# Autodesk Inventor assembly: 000 Ensamblaje hw_DAA - PCB Sensor
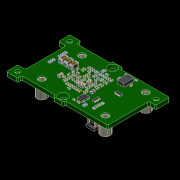
[picture p0: Inventor's stored thumbnail of the model, 180x180]
Saved by Autodesk Inventor 2018 (Build 220112000, 112)
## iProperties
Created: 2024-03-13
Part Number: 000 Ensamblaje hw_DAA - PCB Sensor
Document SubType Name: Assembly
Designer: cda1
Author: cda1
## Documents named in this file (15)
- C:\Users\cda1\Git\DAA\items\hw_DAA\variants\BASIC\3d\000 Ensamblaje hw_DAA - PCB Sensor.iam
- C:\Users\cda1\Git\DAA\items\hw_DAA\3d\hw_DAA - PCB Sensor.ipt
- C:\Users\cda1\Git\DAA\items\_accessories\Componentes PCB\Resistencias\3d_Panasonic\3d\ERJ-2RKF1002X.ipt
- C:\Users\cda1\Git\DAA\items\_accessories\Componentes PCB\Capacitadores\3d_TDK\3d\CGA2B3X7R1H104K050BD.ipt
- C:\Users\cda1\Git\DAA\items\_accessories\Componentes PCB\Condensadores\3d-Murata\3d\GRT188R61C106KE13D\GRT188R61C106KE13D.ipt
- C:\Users\cda1\Git\DAA\items\_accessories\Sensores imagen\3d_Sony\3d\IMX296LQR-C\IMX296LQR-C.ipt
- C:\Users\cda1\Git\DAA\items\_accessories\Componentes PCB\IMU\3d_Bosch\3d\BMI088.ipt
- C:\Users\cda1\Git\DAA\items\_accessories\Componentes PCB\Capacitadores\3d_Murata Electronics\3d\GRT31CC81C226KE01L.ipt
- C:\Users\cda1\Git\DAA\items\_accessories\Componentes PCB\Clock\3d_SiTime\3d\SiT8008BI-22-18E-37.125000G\SiT8008BI-22-18E-37.125000G.ipt
- C:\Users\cda1\Git\DAA\items\_accessories\Componentes PCB\Capacitadores\3d_Murata Electronics\3d\GRT188C81A106ME13D.ipt
- C:\Users\cda1\Git\DAA\items\_accessories\Componentes PCB\Resistencias\3d_Genérico\RESC-0402.ipt
- C:\Users\cda1\Git\DAA\items\_accessories\Componentes PCB\Resistencias\3d_Panasonic\3d\ERJ-2GE0R00X.ipt
- C:\Users\cda1\Git\DAA\items\_accessories\Componentes PCB\Elementos mecanicos soldables\3d_Wurth Electronics\3d\WA-SMST\9774050943\9774050943.ipt
- C:\Users\cda1\Git\DAA\items\_accessories\Componentes PCB\Conectores\3d_Amphenol Communications\SFW15S-2STE1LF\SFW15S-2STE1LF.ipt
- C:\Users\cda1\Git\DAA\items\_accessories\Componentes PCB\Diodos\3d_ST Microelectronics\HSP051-4M10\HSP051-4M10.ipt
## Components (113 placed, 14 different names)
1. hw_DAA - PCB Sensor:1 — Coincidencia:6, Coincidencia:7, Coincidencia:8, Coincidencia:9, Coincidencia:10, Coincidencia:11, Coincidencia:12, Coincidencia:13, Coincidencia:14, Coincidencia:15, Coincidencia:16, Coincidencia:17, Coincidencia:18, Coincidencia:19, Coincidencia:20, Coincidencia:21, Coincidencia:22, Coincidencia:23, Coincidencia:24, Coincidencia:25, Coincidencia:26, Coincidencia:27, Coincidencia:28, Coincidencia:29, Coincidencia:30, Coincidencia:32, Coincidencia:33, Coincidencia:34, Coincidencia:35, Coincidencia:36, Coincidencia:37, Coincidencia:38, Coincidencia:39, Coincidencia:40, Coincidencia:41, Coincidencia:42, Coincidencia:43, Coincidencia:44, Coincidencia:45, Coincidencia:46, Coincidencia:47, Coincidencia:48, Coincidencia:49, Coincidencia:50, Coincidencia:51, Coincidencia:52, Coincidencia:53, Coincidencia:54, Coincidencia:55, Coincidencia:56, Coincidencia:57, Coincidencia:58, Coincidencia:59, Coincidencia:60, Coincidencia:61, Coincidencia:62, Coincidencia:63, Coincidencia:64, Coincidencia:65, Coincidencia:66, Coincidencia:67, Coincidencia:68, Coincidencia:71, Coincidencia:72, Coincidencia:73, Coincidencia:74, Coincidencia:75, Coincidencia:76, Coincidencia:77, Coincidencia:78, Coincidencia:79, Coincidencia:80, Coincidencia:81, Coincidencia:82, Coincidencia:84, Coincidencia:85, Coincidencia:86, Coincidencia:87, Coincidencia:88, Coincidencia:90, Coincidencia:91, Coincidencia:92, Coincidencia:93, Coincidencia:94, Coincidencia:95, Coincidencia:96, Coincidencia:97, Coincidencia:98, Coincidencia:99, Coincidencia:100, Coincidencia:101, Coincidencia:102, Coincidencia:103, Coincidencia:104, Coincidencia:105, Coincidencia:106, Coincidencia:107, Coincidencia:108, Coincidencia:111, Coincidencia:112, Coincidencia:113, Coincidencia:114, Coincidencia:116, Coincidencia:117, Coincidencia:118, Coincidencia:121, Coincidencia:122, Coincidencia:123, Coincidencia:124, Coincidencia:125, Coincidencia:126, Coincidencia:127, Coincidencia:128, Ángulo:3, Ángulo:5, Ángulo:6, Ángulo:7, Ángulo:8, Coincidencia:129, Ángulo:9, Coincidencia:130, Coincidencia:131, Ángulo:10
2. ERJ-2RKF1002X:1 — Coincidencia:6
3. ERJ-2RKF1002X:2 — Coincidencia:7
4. ERJ-2RKF1002X:3 — Coincidencia:18
5. ERJ-2RKF1002X:4 — Coincidencia:17
6. ERJ-2RKF1002X:5 — Coincidencia:16
7. ERJ-2RKF1002X:6 — Coincidencia:15
8. ERJ-2RKF1002X:7 — Coincidencia:14
9. ERJ-2RKF1002X:8 — Coincidencia:13
10. ERJ-2RKF1002X:9 — Coincidencia:12
11. ERJ-2RKF1002X:10 — Coincidencia:11
12. ERJ-2RKF1002X:11 — Coincidencia:10
13. ERJ-2RKF1002X:12 — Coincidencia:9
14. ERJ-2RKF1002X:13 — Coincidencia:8
15. ERJ-2RKF1002X:14 — Coincidencia:19
16. CGA2B3X7R1H104K050BD:1 — Coincidencia:20, Ángulo:6
17. CGA2B3X7R1H104K050BD:2 — Coincidencia:21, Ángulo:7
18. CGA2B3X7R1H104K050BD:3 — Coincidencia:22
19. CGA2B3X7R1H104K050BD:4 — Coincidencia:23, Ángulo:5
20. CGA2B3X7R1H104K050BD:5 — Coincidencia:24
21. CGA2B3X7R1H104K050BD:6 — Coincidencia:25
22. CGA2B3X7R1H104K050BD:7 — Coincidencia:26
23. CGA2B3X7R1H104K050BD:8 — Coincidencia:28
24. CGA2B3X7R1H104K050BD:9 — Coincidencia:29
25. CGA2B3X7R1H104K050BD:10 — Coincidencia:30, Ángulo:8
26. CGA2B3X7R1H104K050BD:11 — Coincidencia:27
27. CGA2B3X7R1H104K050BD:13 — Coincidencia:32
28. CGA2B3X7R1H104K050BD:14 — Coincidencia:33
29. CGA2B3X7R1H104K050BD:15 — Coincidencia:34
30. CGA2B3X7R1H104K050BD:16 — Coincidencia:35
31. CGA2B3X7R1H104K050BD:17 — Coincidencia:36
32. CGA2B3X7R1H104K050BD:18 — Coincidencia:37
33. CGA2B3X7R1H104K050BD:19 — Coincidencia:38
34. CGA2B3X7R1H104K050BD:20 — Coincidencia:39
35. CGA2B3X7R1H104K050BD:21 — Coincidencia:40
36. CGA2B3X7R1H104K050BD:22 — Coincidencia:41
37. CGA2B3X7R1H104K050BD:23 — Coincidencia:42
38. CGA2B3X7R1H104K050BD:24 — Coincidencia:43
39. CGA2B3X7R1H104K050BD:25 — Coincidencia:44
40. CGA2B3X7R1H104K050BD:26 — Coincidencia:45
41. CGA2B3X7R1H104K050BD:27 — Coincidencia:46
42. CGA2B3X7R1H104K050BD:28 — Coincidencia:47
43. CGA2B3X7R1H104K050BD:29 — Coincidencia:48
44. CGA2B3X7R1H104K050BD:30 — Coincidencia:51
45. CGA2B3X7R1H104K050BD:31 — Coincidencia:52
46. CGA2B3X7R1H104K050BD:32 — Coincidencia:53
47. CGA2B3X7R1H104K050BD:33 — Coincidencia:68
48. CGA2B3X7R1H104K050BD:34 — Coincidencia:67
49. CGA2B3X7R1H104K050BD:35 — Coincidencia:66
50. CGA2B3X7R1H104K050BD:38 — Coincidencia:62
51. CGA2B3X7R1H104K050BD:39 — Coincidencia:63
52. CGA2B3X7R1H104K050BD:40 — Coincidencia:64
53. CGA2B3X7R1H104K050BD:41 — Coincidencia:65
54. CGA2B3X7R1H104K050BD:42 — Coincidencia:61
55. CGA2B3X7R1H104K050BD:43 — Coincidencia:60
56. CGA2B3X7R1H104K050BD:44 — Coincidencia:59
57. CGA2B3X7R1H104K050BD:45 — Coincidencia:58
58. CGA2B3X7R1H104K050BD:46 — Coincidencia:54
59. CGA2B3X7R1H104K050BD:47 — Coincidencia:55
60. CGA2B3X7R1H104K050BD:48 — Coincidencia:49
61. CGA2B3X7R1H104K050BD:49 — Coincidencia:50
62. CGA2B3X7R1H104K050BD:50 — Coincidencia:56
63. CGA2B3X7R1H104K050BD:51 — Coincidencia:57
64. CGA2B3X7R1H104K050BD:52 — Coincidencia:71
65. CGA2B3X7R1H104K050BD:53 — Coincidencia:72
66. CGA2B3X7R1H104K050BD:54 — Coincidencia:73
67. CGA2B3X7R1H104K050BD:55 — Coincidencia:74
68. CGA2B3X7R1H104K050BD:56 — Coincidencia:75
69. CGA2B3X7R1H104K050BD:57 — Coincidencia:76
70. CGA2B3X7R1H104K050BD:58 — Coincidencia:77
71. CGA2B3X7R1H104K050BD:59 — Coincidencia:78
72. GRT188R61C106KE13D:1 — Coincidencia:79
73. GRT188R61C106KE13D:2 — Coincidencia:80
74. GRT188R61C106KE13D:3 — Coincidencia:81
75. GRT188R61C106KE13D:4 — Coincidencia:82
76. IMX296LQR-C:1 — Coincidencia:84
77. BMI088:1 — Coincidencia:85
78. GRT31CC81C226KE01L:1 — Coincidencia:86
79. GRT31CC81C226KE01L:2 — Coincidencia:87
80. SiT8008BI-22-18E-37.125000G:1 — Coincidencia:88
81. ERJ-2RKF1002X:16 — Coincidencia:90, Ángulo:1
82. ERJ-2RKF1002X:17 — Coincidencia:91, Ángulo:1, Ángulo:2
83. ERJ-2RKF1002X:18 — Coincidencia:92, Ángulo:2
84. ERJ-2RKF1002X:19 — Coincidencia:94
85. ERJ-2RKF1002X:20 — Coincidencia:93
86. CGA2B3X7R1H104K050BD:60 — Coincidencia:95
87. CGA2B3X7R1H104K050BD:61 — Coincidencia:96
88. CGA2B3X7R1H104K050BD:62 — Coincidencia:97
89. GRT188C81A106ME13D:1 — Coincidencia:98
90. GRT31CC81C226KE01L:3 — Coincidencia:99, Ángulo:3
91. ERJ-2RKF1002X:21 — Coincidencia:100
92. ERJ-2RKF1002X:22 — Coincidencia:101
93. CGA2B3X7R1H104K050BD:63 — Coincidencia:102
94. CGA2B3X7R1H104K050BD:64 — Coincidencia:103
95. RESC-0402:1 — Coincidencia:104
96. ERJ-2GE0R00X:1 — Coincidencia:105
97. RESC-0402:2 — Coincidencia:106
98. CGA2B3X7R1H104K050BD:65 — Coincidencia:108
99. CGA2B3X7R1H104K050BD:66 — Coincidencia:107
100. ERJ-2RKF1002X:25 — Coincidencia:118
101. ERJ-2RKF1002X:26 — Coincidencia:117
102. ERJ-2RKF1002X:27 — Coincidencia:116
103. ERJ-2RKF1002X:29 — Coincidencia:114
104. ERJ-2RKF1002X:30 — Coincidencia:113
105. ERJ-2RKF1002X:31 — Coincidencia:112
106. ERJ-2RKF1002X:32 — Coincidencia:111
107. 9774050943:1 — Coincidencia:123, Coincidencia:124
108. 9774050943:2 — Coincidencia:121, Coincidencia:125
109. 9774050943:3 — Coincidencia:122, Coincidencia:126
110. 9774050943:4 — Coincidencia:127, Coincidencia:128
111. SFW15S-2STE1LF:1 — Coincidencia:129, Ángulo:9
112. HSP051-4M10:1 — Coincidencia:130
113. HSP051-4M10:2 — Coincidencia:131, Ángulo:10
## Relationships (125: Mate 116, Angle 9)
- Coincidencia:6 [Mate]: hw_DAA - PCB Sensor:1 ↔ ERJ-2RKF1002X:1
- Coincidencia:7 [Mate]: hw_DAA - PCB Sensor:1 ↔ ERJ-2RKF1002X:2
- Coincidencia:8 [Mate]: hw_DAA - PCB Sensor:1 ↔ ERJ-2RKF1002X:13
- Coincidencia:9 [Mate]: hw_DAA - PCB Sensor:1 ↔ ERJ-2RKF1002X:12
- Coincidencia:10 [Mate]: hw_DAA - PCB Sensor:1 ↔ ERJ-2RKF1002X:11
- Coincidencia:11 [Mate]: hw_DAA - PCB Sensor:1 ↔ ERJ-2RKF1002X:10
- Coincidencia:12 [Mate]: hw_DAA - PCB Sensor:1 ↔ ERJ-2RKF1002X:9
- Coincidencia:13 [Mate]: hw_DAA - PCB Sensor:1 ↔ ERJ-2RKF1002X:8
- Coincidencia:14 [Mate]: hw_DAA - PCB Sensor:1 ↔ ERJ-2RKF1002X:7
- Coincidencia:15 [Mate]: hw_DAA - PCB Sensor:1 ↔ ERJ-2RKF1002X:6
- Coincidencia:16 [Mate]: hw_DAA - PCB Sensor:1 ↔ ERJ-2RKF1002X:5
- Coincidencia:17 [Mate]: hw_DAA - PCB Sensor:1 ↔ ERJ-2RKF1002X:4
- Coincidencia:18 [Mate]: hw_DAA - PCB Sensor:1 ↔ ERJ-2RKF1002X:3
- Coincidencia:19 [Mate]: hw_DAA - PCB Sensor:1 ↔ ERJ-2RKF1002X:14
- Coincidencia:20 [Mate]: hw_DAA - PCB Sensor:1 ↔ CGA2B3X7R1H104K050BD:1
- Coincidencia:21 [Mate]: hw_DAA - PCB Sensor:1 ↔ CGA2B3X7R1H104K050BD:2
- Coincidencia:22 [Mate]: hw_DAA - PCB Sensor:1 ↔ CGA2B3X7R1H104K050BD:3
- Coincidencia:23 [Mate]: hw_DAA - PCB Sensor:1 ↔ CGA2B3X7R1H104K050BD:4
- Coincidencia:24 [Mate]: hw_DAA - PCB Sensor:1 ↔ CGA2B3X7R1H104K050BD:5
- Coincidencia:25 [Mate]: hw_DAA - PCB Sensor:1 ↔ CGA2B3X7R1H104K050BD:6
- Coincidencia:26 [Mate]: hw_DAA - PCB Sensor:1 ↔ CGA2B3X7R1H104K050BD:7
- Coincidencia:27 [Mate]: hw_DAA - PCB Sensor:1 ↔ CGA2B3X7R1H104K050BD:11
- Coincidencia:28 [Mate]: hw_DAA - PCB Sensor:1 ↔ CGA2B3X7R1H104K050BD:8
- Coincidencia:29 [Mate]: hw_DAA - PCB Sensor:1 ↔ CGA2B3X7R1H104K050BD:9
- Coincidencia:30 [Mate]: hw_DAA - PCB Sensor:1 ↔ CGA2B3X7R1H104K050BD:10
- Coincidencia:32 [Mate]: hw_DAA - PCB Sensor:1 ↔ CGA2B3X7R1H104K050BD:13
- Coincidencia:33 [Mate]: hw_DAA - PCB Sensor:1 ↔ CGA2B3X7R1H104K050BD:14
- Coincidencia:34 [Mate]: hw_DAA - PCB Sensor:1 ↔ CGA2B3X7R1H104K050BD:15
- Coincidencia:35 [Mate]: hw_DAA - PCB Sensor:1 ↔ CGA2B3X7R1H104K050BD:16
- Coincidencia:36 [Mate]: hw_DAA - PCB Sensor:1 ↔ CGA2B3X7R1H104K050BD:17
- Coincidencia:37 [Mate]: hw_DAA - PCB Sensor:1 ↔ CGA2B3X7R1H104K050BD:18
- Coincidencia:38 [Mate]: hw_DAA - PCB Sensor:1 ↔ CGA2B3X7R1H104K050BD:19
- Coincidencia:39 [Mate]: hw_DAA - PCB Sensor:1 ↔ CGA2B3X7R1H104K050BD:20
- Coincidencia:40 [Mate]: hw_DAA - PCB Sensor:1 ↔ CGA2B3X7R1H104K050BD:21
- Coincidencia:41 [Mate]: hw_DAA - PCB Sensor:1 ↔ CGA2B3X7R1H104K050BD:22
- Coincidencia:42 [Mate]: hw_DAA - PCB Sensor:1 ↔ CGA2B3X7R1H104K050BD:23
- Coincidencia:43 [Mate]: hw_DAA - PCB Sensor:1 ↔ CGA2B3X7R1H104K050BD:24
- Coincidencia:44 [Mate]: hw_DAA - PCB Sensor:1 ↔ CGA2B3X7R1H104K050BD:25
- Coincidencia:45 [Mate]: hw_DAA - PCB Sensor:1 ↔ CGA2B3X7R1H104K050BD:26
- Coincidencia:46 [Mate]: hw_DAA - PCB Sensor:1 ↔ CGA2B3X7R1H104K050BD:27
- Coincidencia:47 [Mate]: hw_DAA - PCB Sensor:1 ↔ CGA2B3X7R1H104K050BD:28
- Coincidencia:48 [Mate]: hw_DAA - PCB Sensor:1 ↔ CGA2B3X7R1H104K050BD:29
- Coincidencia:49 [Mate]: hw_DAA - PCB Sensor:1 ↔ CGA2B3X7R1H104K050BD:48
- Coincidencia:50 [Mate]: hw_DAA - PCB Sensor:1 ↔ CGA2B3X7R1H104K050BD:49
- Coincidencia:51 [Mate]: hw_DAA - PCB Sensor:1 ↔ CGA2B3X7R1H104K050BD:30
- Coincidencia:52 [Mate]: hw_DAA - PCB Sensor:1 ↔ CGA2B3X7R1H104K050BD:31
- Coincidencia:53 [Mate]: hw_DAA - PCB Sensor:1 ↔ CGA2B3X7R1H104K050BD:32
- Coincidencia:54 [Mate]: hw_DAA - PCB Sensor:1 ↔ CGA2B3X7R1H104K050BD:46
- Coincidencia:55 [Mate]: hw_DAA - PCB Sensor:1 ↔ CGA2B3X7R1H104K050BD:47
- Coincidencia:56 [Mate]: hw_DAA - PCB Sensor:1 ↔ CGA2B3X7R1H104K050BD:50
- Coincidencia:57 [Mate]: hw_DAA - PCB Sensor:1 ↔ CGA2B3X7R1H104K050BD:51
- Coincidencia:58 [Mate]: hw_DAA - PCB Sensor:1 ↔ CGA2B3X7R1H104K050BD:45
- Coincidencia:59 [Mate]: hw_DAA - PCB Sensor:1 ↔ CGA2B3X7R1H104K050BD:44
- Coincidencia:60 [Mate]: hw_DAA - PCB Sensor:1 ↔ CGA2B3X7R1H104K050BD:43
- Coincidencia:61 [Mate]: hw_DAA - PCB Sensor:1 ↔ CGA2B3X7R1H104K050BD:42
- Coincidencia:62 [Mate]: hw_DAA - PCB Sensor:1 ↔ CGA2B3X7R1H104K050BD:38
- Coincidencia:63 [Mate]: hw_DAA - PCB Sensor:1 ↔ CGA2B3X7R1H104K050BD:39
- Coincidencia:64 [Mate]: hw_DAA - PCB Sensor:1 ↔ CGA2B3X7R1H104K050BD:40
- Coincidencia:65 [Mate]: hw_DAA - PCB Sensor:1 ↔ CGA2B3X7R1H104K050BD:41
- Coincidencia:66 [Mate]: hw_DAA - PCB Sensor:1 ↔ CGA2B3X7R1H104K050BD:35
- Coincidencia:67 [Mate]: hw_DAA - PCB Sensor:1 ↔ CGA2B3X7R1H104K050BD:34
- Coincidencia:68 [Mate]: hw_DAA - PCB Sensor:1 ↔ CGA2B3X7R1H104K050BD:33
- Coincidencia:71 [Mate]: hw_DAA - PCB Sensor:1 ↔ CGA2B3X7R1H104K050BD:52
- Coincidencia:72 [Mate]: hw_DAA - PCB Sensor:1 ↔ CGA2B3X7R1H104K050BD:53
- Coincidencia:73 [Mate]: hw_DAA - PCB Sensor:1 ↔ CGA2B3X7R1H104K050BD:54
- Coincidencia:74 [Mate]: hw_DAA - PCB Sensor:1 ↔ CGA2B3X7R1H104K050BD:55
- Coincidencia:75 [Mate]: hw_DAA - PCB Sensor:1 ↔ CGA2B3X7R1H104K050BD:56
- Coincidencia:76 [Mate]: hw_DAA - PCB Sensor:1 ↔ CGA2B3X7R1H104K050BD:57
- Coincidencia:77 [Mate]: hw_DAA - PCB Sensor:1 ↔ CGA2B3X7R1H104K050BD:58
- Coincidencia:78 [Mate]: hw_DAA - PCB Sensor:1 ↔ CGA2B3X7R1H104K050BD:59
- Coincidencia:79 [Mate]: hw_DAA - PCB Sensor:1 ↔ GRT188R61C106KE13D:1
- Coincidencia:80 [Mate]: hw_DAA - PCB Sensor:1 ↔ GRT188R61C106KE13D:2
- Coincidencia:81 [Mate]: hw_DAA - PCB Sensor:1 ↔ GRT188R61C106KE13D:3
- Coincidencia:82 [Mate]: hw_DAA - PCB Sensor:1 ↔ GRT188R61C106KE13D:4
- Coincidencia:84 [Mate]: hw_DAA - PCB Sensor:1 ↔ IMX296LQR-C:1
- Coincidencia:85 [Mate]: hw_DAA - PCB Sensor:1 ↔ BMI088:1
- Coincidencia:86 [Mate]: hw_DAA - PCB Sensor:1 ↔ GRT31CC81C226KE01L:1
- Coincidencia:87 [Mate]: hw_DAA - PCB Sensor:1 ↔ GRT31CC81C226KE01L:2
- Coincidencia:88 [Mate]: hw_DAA - PCB Sensor:1 ↔ SiT8008BI-22-18E-37.125000G:1
- Coincidencia:90 [Mate]: hw_DAA - PCB Sensor:1 ↔ ERJ-2RKF1002X:16
- Coincidencia:91 [Mate]: hw_DAA - PCB Sensor:1 ↔ ERJ-2RKF1002X:17
- Coincidencia:92 [Mate]: hw_DAA - PCB Sensor:1 ↔ ERJ-2RKF1002X:18
- Coincidencia:93 [Mate]: hw_DAA - PCB Sensor:1 ↔ ERJ-2RKF1002X:20
- Coincidencia:94 [Mate]: hw_DAA - PCB Sensor:1 ↔ ERJ-2RKF1002X:19
- Coincidencia:95 [Mate]: hw_DAA - PCB Sensor:1 ↔ CGA2B3X7R1H104K050BD:60
- Coincidencia:96 [Mate]: hw_DAA - PCB Sensor:1 ↔ CGA2B3X7R1H104K050BD:61
- Coincidencia:97 [Mate]: hw_DAA - PCB Sensor:1 ↔ CGA2B3X7R1H104K050BD:62
- Coincidencia:98 [Mate]: hw_DAA - PCB Sensor:1 ↔ GRT188C81A106ME13D:1
- Coincidencia:99 [Mate]: hw_DAA - PCB Sensor:1 ↔ GRT31CC81C226KE01L:3
- Coincidencia:100 [Mate]: hw_DAA - PCB Sensor:1 ↔ ERJ-2RKF1002X:21
- Coincidencia:101 [Mate]: hw_DAA - PCB Sensor:1 ↔ ERJ-2RKF1002X:22
- Coincidencia:102 [Mate]: hw_DAA - PCB Sensor:1 ↔ CGA2B3X7R1H104K050BD:63
- Coincidencia:103 [Mate]: hw_DAA - PCB Sensor:1 ↔ CGA2B3X7R1H104K050BD:64
- Coincidencia:104 [Mate]: hw_DAA - PCB Sensor:1 ↔ RESC-0402:1
- Coincidencia:105 [Mate]: hw_DAA - PCB Sensor:1 ↔ ERJ-2GE0R00X:1
- Coincidencia:106 [Mate]: hw_DAA - PCB Sensor:1 ↔ RESC-0402:2
- Coincidencia:107 [Mate]: hw_DAA - PCB Sensor:1 ↔ CGA2B3X7R1H104K050BD:66
- Coincidencia:108 [Mate]: hw_DAA - PCB Sensor:1 ↔ CGA2B3X7R1H104K050BD:65
- Coincidencia:111 [Mate]: hw_DAA - PCB Sensor:1 ↔ ERJ-2RKF1002X:32
- Coincidencia:112 [Mate]: hw_DAA - PCB Sensor:1 ↔ ERJ-2RKF1002X:31
- Coincidencia:113 [Mate]: hw_DAA - PCB Sensor:1 ↔ ERJ-2RKF1002X:30
- Coincidencia:114 [Mate]: hw_DAA - PCB Sensor:1 ↔ ERJ-2RKF1002X:29
- Coincidencia:116 [Mate]: hw_DAA - PCB Sensor:1 ↔ ERJ-2RKF1002X:27
- Coincidencia:117 [Mate]: hw_DAA - PCB Sensor:1 ↔ ERJ-2RKF1002X:26
- Coincidencia:118 [Mate]: hw_DAA - PCB Sensor:1 ↔ ERJ-2RKF1002X:25
- Coincidencia:121 [Mate]: hw_DAA - PCB Sensor:1 ↔ 9774050943:2
- Coincidencia:122 [Mate]: hw_DAA - PCB Sensor:1 ↔ 9774050943:3
- Coincidencia:123 [Mate]: hw_DAA - PCB Sensor:1 ↔ 9774050943:1
- Coincidencia:124 [Mate]: hw_DAA - PCB Sensor:1 ↔ 9774050943:1
- Coincidencia:125 [Mate]: hw_DAA - PCB Sensor:1 ↔ 9774050943:2
- Coincidencia:126 [Mate]: hw_DAA - PCB Sensor:1 ↔ 9774050943:3
- Ángulo:1 [Angle] (0 deg): ERJ-2RKF1002X:16 ↔ ERJ-2RKF1002X:17
- Ángulo:2 [Angle] (0 deg): ERJ-2RKF1002X:17 ↔ ERJ-2RKF1002X:18
- Coincidencia:127 [Mate]: hw_DAA - PCB Sensor:1 ↔ 9774050943:4
- Coincidencia:128 [Mate]: hw_DAA - PCB Sensor:1 ↔ 9774050943:4
- Ángulo:3 [Angle] (0 deg): hw_DAA - PCB Sensor:1 ↔ GRT31CC81C226KE01L:3
- Ángulo:5 [Angle] (0 deg): hw_DAA - PCB Sensor:1 ↔ CGA2B3X7R1H104K050BD:4
- Ángulo:6 [Angle] (0 deg): hw_DAA - PCB Sensor:1 ↔ CGA2B3X7R1H104K050BD:1
- Ángulo:7 [Angle] (0 deg): hw_DAA - PCB Sensor:1 ↔ CGA2B3X7R1H104K050BD:2
- Ángulo:8 [Angle] (0 deg): hw_DAA - PCB Sensor:1 ↔ CGA2B3X7R1H104K050BD:10
- Coincidencia:129 [Mate]: hw_DAA - PCB Sensor:1 ↔ SFW15S-2STE1LF:1
- Ángulo:9 [Angle] (0 deg): hw_DAA - PCB Sensor:1 ↔ SFW15S-2STE1LF:1
- Coincidencia:130 [Mate]: hw_DAA - PCB Sensor:1 ↔ HSP051-4M10:1
- Coincidencia:131 [Mate]: hw_DAA - PCB Sensor:1 ↔ HSP051-4M10:2
- Ángulo:10 [Angle] (0 deg): hw_DAA - PCB Sensor:1 ↔ HSP051-4M10:2
